# Autodesk Inventor assembly: Catapult
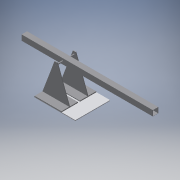
[picture p0: Inventor's stored thumbnail of the model, 180x180]
Saved by Autodesk Inventor 2016 SP1 (Build 200210100, 210)
## iProperties
Created: 2016-01-12
Part Number: Catapult
Document SubType Name: Assembly
Designer: steele
Author: steele
## Documents named in this file (5)
- C:\snobotics\CAD-Development\robSteele\SnoBotics2016\FirstCutCatapult\Catapult.iam
- C:\snobotics\CAD-Development\robSteele\SnoBotics2016\FirstCutCatapult\CatapultBase.ipt
- C:\snobotics\CAD-Development\robSteele\SnoBotics2016\FirstCutCatapult\CatapultSupport.ipt
- C:\snobotics\CAD-Development\robSteele\SnoBotics2016\FirstCutCatapult\CatapultAxel.ipt
- C:\snobotics\CAD-Development\robSteele\SnoBotics2016\FirstCutCatapult\catapultArm.ipt
## Components (5 placed, 4 different names)
1. CatapultBase:1 — Mate:1, Flush:1, Mate:2, Mate:3, Flush:2, Mate:4
2. CatapultSupport:1 — Mate:1, Flush:1, Mate:2, Insert:1
3. CatapultSupport:2 — Mate:3, Flush:2, Mate:4
4. CatapultAxel:1 — Insert:1, Mate:5
5. catapultArm:1 — Mate:5, Mate:6
## Relationships (9: Mate 6, Flush 2, Insert 1)
- Mate:1: CatapultBase:1 ↔ CatapultSupport:1
- Flush:1: CatapultBase:1 ↔ CatapultSupport:1
- Mate:2: CatapultBase:1 ↔ CatapultSupport:1
- Mate:3: CatapultBase:1 ↔ CatapultSupport:2
- Flush:2: CatapultBase:1 ↔ CatapultSupport:2
- Mate:4: CatapultBase:1 ↔ CatapultSupport:2
- Insert:1: CatapultSupport:1 ↔ CatapultAxel:1
- Mate:5: CatapultAxel:1 ↔ catapultArm:1
- Mate:6: catapultArm:1
